# Autodesk Inventor assembly: Assembly_Cube_Seeed_Xiao_Sense_Camera
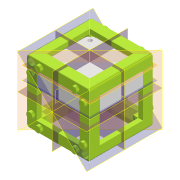
[picture p0: Inventor's stored thumbnail of the model, 180x180]
Saved by Autodesk Inventor 2022 (Build 260153000, 153)
## iProperties
Created: 2023-05-29
Part Number: Assembly_Cube_Seeed_Xiao_Sense_Camera
Document SubType Name: Assembly
Designer: diederichbenedict
Author: diederichbenedict
## Documents named in this file (3)
- C:\Users\diederichbenedict\Dropbox\Dokumente\Promotion\PROJECTS\openUC2-CAD\INVENTOR\Assembly_Cube_Seeed_Xiao_Sense_Camera.iam
- C:\Users\diederichbenedict\Dropbox\Dokumente\Promotion\PROJECTS\openUC2-CAD\INVENTOR\Assembly_Cube_empty_IM_v3.iam
- C:\Users\diederichbenedict\Dropbox\Dokumente\Promotion\PROJECTS\openUC2-CAD\INVENTOR\Assembly_Cube_SEEED_Xiao_Sense_Camera_v3.iam
## Components (2 placed, 2 different names)
1. Assembly_Cube_empty_IM_v3:1 [sub-assembly] — Passend:1, Passend:2, Winkel:1
2. Assembly_Cube_SEEED_Xiao_Sense_Camera_v3:1 [sub-assembly] — Passend:1, Passend:2, Winkel:1
## Relationships (3: Mate 2, Angle 1)
- Passend:1 [Mate]: Assembly_Cube_empty_IM_v3:1 ↔ Assembly_Cube_SEEED_Xiao_Sense_Camera_v3:1
- Passend:2 [Mate]: Assembly_Cube_empty_IM_v3:1 ↔ Assembly_Cube_SEEED_Xiao_Sense_Camera_v3:1
- Winkel:1 [Angle] (0 deg): Assembly_Cube_empty_IM_v3:1 ↔ Assembly_Cube_SEEED_Xiao_Sense_Camera_v3:1
